# Autodesk Inventor assembly: rubber band holder
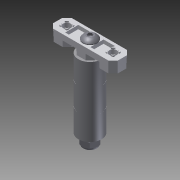
[picture p0: Inventor's stored thumbnail of the model, 180x180]
Saved by Autodesk Inventor 2014 SP1 (Build 180222100, 222)
## iProperties
Created: 2014-04-04
Part Number: rubber band holder
Document SubType Name: Assembly
Designer: Ryan
Author: Ryan
## Documents named in this file (5)
- C:\Users\Ryan\Desktop\sw\toss up 5th A bot\intake\rubber band holder.iam
- C:\Users\Ryan\Desktop\sw\lib\Aperture VEX CAD Library\Spacers\SPACER-0500-0500.ipt
- C:\Users\Ryan\Desktop\sw\lib\Aperture VEX CAD Library\Bearing Blocks\Bearing Block.ipt
- C:\Users\Ryan\Desktop\sw\lib\Aperture VEX CAD Library\Hardware\8-32\8-32_.500.ipt
- C:\Users\Ryan\Desktop\sw\lib\Aperture VEX CAD Library\Hardware\8-32\8-32 nylock.ipt
## Components (6 placed, 4 different names)
1. SPACER-0500-0500:1 — Mate:1, Mate:2, Mate:9, Mate:10
2. SPACER-0500-0500:2 — Mate:1, Mate:2, Mate:3, Mate:4
3. SPACER-0500-0500:3 — Mate:3, Mate:4, Mate:5, Mate:6
4. Bearing Block:1 — Mate:5, Mate:6, Mate:7, Mate:8
5. 8-32_.500:1 — Mate:7, Mate:8
6. 8-32 nylock:1 — Mate:9, Mate:10
## Relationships (10: Mate 10)
- Mate:1: SPACER-0500-0500:1 ↔ SPACER-0500-0500:2
- Mate:2: SPACER-0500-0500:1 ↔ SPACER-0500-0500:2
- Mate:3: SPACER-0500-0500:2 ↔ SPACER-0500-0500:3
- Mate:4: SPACER-0500-0500:2 ↔ SPACER-0500-0500:3
- Mate:5: SPACER-0500-0500:3 ↔ Bearing Block:1
- Mate:6: SPACER-0500-0500:3 ↔ Bearing Block:1
- Mate:7: Bearing Block:1 ↔ 8-32_.500:1
- Mate:8: Bearing Block:1 ↔ 8-32_.500:1
- Mate:9: SPACER-0500-0500:1 ↔ 8-32 nylock:1
- Mate:10 (1.1684 mm): SPACER-0500-0500:1 ↔ 8-32 nylock:1
